# Autodesk Inventor assembly: OuterFrameInternals
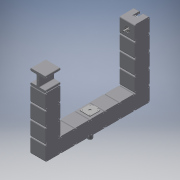
[picture p0: Inventor's stored thumbnail of the model, 180x180]
Saved by Autodesk Inventor 2016 (Build 200138000, 138)
## iProperties
Created: 2016-05-22
Part Number: OuterFrameInternals
Document SubType Name: Assembly
Designer: Kurtis
Author: Kurtis
## Documents named in this file (6)
- C:\Users\Kurtis\Git\CAD\Sentry Camera\cad\OuterFrameInternals.iam
- C:\Users\Kurtis\Git\CAD\Sentry Camera\cad\60x60Motor.ipt
- C:\Users\Kurtis\Git\CAD\Sentry Camera\cad\assets\SmallStepper.ipt
- C:\Users\Kurtis\Git\CAD\Sentry Camera\cad\MotorTripodCoupler.ipt
- C:\Users\Kurtis\Git\CAD\Sentry Camera\cad\60x60Spacer.ipt
- C:\Users\Kurtis\Git\CAD\Sentry Camera\cad\60x60IdlerNoMotor.ipt
## Components (18 placed, 5 different names)
1. 60x60Motor:1 — Cylindrical:1, Flush:1, Flush:2, Mate:1, Flush:7, Mate:4
2. SmallStepper:1 — Cylindrical:1, Cylindrical:2
3. MotorTripodCoupler:1 — Cylindrical:2
4. 60x60Spacer:1 — Flush:1, Flush:2, Flush:3, Flush:4, Mate:1, Mate:2, Flush:8
5. 60x60Spacer:2 — Flush:3, Flush:4, Flush:5, Flush:6, Mate:2, Mate:3
6. 60x60Spacer:3 — Flush:5, Flush:6, Mate:3, Flush:13, Flush:14, Flush:15, Mate:7, Flush:16
7. 60x60Spacer:4 — Flush:7, Flush:8, Flush:9, Flush:10, Mate:4, Mate:5
8. 60x60Spacer:5 — Flush:9, Flush:10, Flush:11, Flush:12, Mate:5, Mate:6
9. 60x60Spacer:6 — Flush:11, Flush:12, Mate:6, Flush:19, Flush:20, Mate:10, Flush:22
10. 60x60Spacer:7 — Flush:13, Mate:7, Mate:8, Flush:16, Flush:17
11. 60x60Spacer:8 — Flush:14, Mate:9, Flush:18, Flush:27, Flush:28, Mate:14
12. 60x60Spacer:9 — Flush:15, Mate:8, Mate:9, Flush:17, Flush:18
13. 60x60Spacer:10 — Flush:19, Mate:10, Mate:11, Flush:22, Flush:23
14. 60x60Spacer:11 — Flush:20, Flush:21, Mate:11, Mate:12, Flush:23, Flush:24
15. 60x60Spacer:12 — Flush:21, Mate:12, Flush:24, Flush:25, Flush:26, Mate:13
16. 60x60Motor:2 — Flush:25, Flush:26, Mate:13, Cylindrical:3
17. 60x60IdlerNoMotor:1 — Flush:27, Flush:28, Mate:14
18. SmallStepper:2 — Cylindrical:3
## Relationships (45: Flush 28, Mate 14, CylindricalJoint 3)
- Cylindrical:1: 60x60Motor:1 ↔ SmallStepper:1
- Cylindrical:2: SmallStepper:1 ↔ MotorTripodCoupler:1
- Flush:1: 60x60Motor:1 ↔ 60x60Spacer:1
- Flush:2: 60x60Motor:1 ↔ 60x60Spacer:1
- Flush:3: 60x60Spacer:1 ↔ 60x60Spacer:2
- Flush:4: 60x60Spacer:1 ↔ 60x60Spacer:2
- Flush:5: 60x60Spacer:2 ↔ 60x60Spacer:3
- Flush:6: 60x60Spacer:2 ↔ 60x60Spacer:3
- Mate:1: 60x60Motor:1 ↔ 60x60Spacer:1
- Mate:2: 60x60Spacer:1 ↔ 60x60Spacer:2
- Mate:3: 60x60Spacer:2 ↔ 60x60Spacer:3
- Flush:7: 60x60Motor:1 ↔ 60x60Spacer:4
- Flush:8: 60x60Spacer:1 ↔ 60x60Spacer:4
- Flush:9: 60x60Spacer:4 ↔ 60x60Spacer:5
- Flush:10: 60x60Spacer:4 ↔ 60x60Spacer:5
- Flush:11: 60x60Spacer:5 ↔ 60x60Spacer:6
- Flush:12: 60x60Spacer:5 ↔ 60x60Spacer:6
- Mate:4: 60x60Motor:1 ↔ 60x60Spacer:4
- Mate:5: 60x60Spacer:4 ↔ 60x60Spacer:5
- Mate:6: 60x60Spacer:5 ↔ 60x60Spacer:6
- Flush:13: 60x60Spacer:3 ↔ 60x60Spacer:7
- Flush:14: 60x60Spacer:3 ↔ 60x60Spacer:8
- Flush:15: 60x60Spacer:3 ↔ 60x60Spacer:9
- Mate:7: 60x60Spacer:3 ↔ 60x60Spacer:7
- Mate:8: 60x60Spacer:7 ↔ 60x60Spacer:9
- Mate:9: 60x60Spacer:8 ↔ 60x60Spacer:9
- Flush:16: 60x60Spacer:3 ↔ 60x60Spacer:7
- Flush:17: 60x60Spacer:7 ↔ 60x60Spacer:9
- Flush:18: 60x60Spacer:8 ↔ 60x60Spacer:9
- Flush:19: 60x60Spacer:6 ↔ 60x60Spacer:10
- Flush:20: 60x60Spacer:6 ↔ 60x60Spacer:11
- Flush:21: 60x60Spacer:11 ↔ 60x60Spacer:12
- Mate:10: 60x60Spacer:6 ↔ 60x60Spacer:10
- Mate:11: 60x60Spacer:10 ↔ 60x60Spacer:11
- Mate:12: 60x60Spacer:11 ↔ 60x60Spacer:12
- Flush:22: 60x60Spacer:6 ↔ 60x60Spacer:10
- Flush:23: 60x60Spacer:10 ↔ 60x60Spacer:11
- Flush:24: 60x60Spacer:11 ↔ 60x60Spacer:12
- Flush:25: 60x60Spacer:12 ↔ 60x60Motor:2
- Flush:26: 60x60Spacer:12 ↔ 60x60Motor:2
- Mate:13: 60x60Spacer:12 ↔ 60x60Motor:2
- Flush:27: 60x60Spacer:8 ↔ 60x60IdlerNoMotor:1
- Flush:28: 60x60Spacer:8 ↔ 60x60IdlerNoMotor:1
- Mate:14: 60x60Spacer:8 ↔ 60x60IdlerNoMotor:1
- Cylindrical:3: 60x60Motor:2 ↔ SmallStepper:2
